# Autodesk Inventor assembly: Assembly1
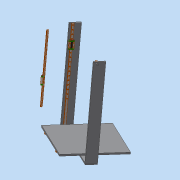
[picture p0: Inventor's stored thumbnail of the model, 180x180]
Saved by Autodesk Inventor 2016 (Build 200138000, 138)
## iProperties
Created: 2017-03-05
Part Number: Assembly1
Document SubType Name: Assembly
Designer: Errrm
Author: Errrm
## Documents named in this file (13)
- C:\Users\Lillahunden\Documents\Inventor\3dprinter\Assembly1.iam
- C:\Users\Lillahunden\Documents\Inventor\3dprinter\bed.ipt
- C:\Users\Lillahunden\Documents\Inventor\3dprinter\sideframe.ipt
- C:\Users\Lillahunden\Documents\Inventor\3dprinter\MGN7z.ipt
- C:\Users\Lillahunden\Documents\Inventor\3dprinter\MGN7x.ipt
- C:\Users\Lillahunden\Documents\Inventor\3dprinter\MGN7y.ipt
- C:\Users\Lillahunden\Documents\Inventor\3dprinter\MGN7-H.ipt
- C:\Users\Lillahunden\Documents\Inventor\3dprinter\bottomplate.ipt
- C:\Users\Lillahunden\Documents\Inventor\3dprinter\flat.ipt
- C:\Users\Lillahunden\Documents\Inventor\3dprinter\Angled foot.ipt
- C:\Users\Lillahunden\Documents\Inventor\3dprinter\Assembly1\Design Accelerator\Bolted Connection1.iam
- C:\Users\Lillahunden\Documents\Inventor\3dprinter\Assembly1\Design Accelerator\Bolted Connection2.iam
- C:\Users\Lillahunden\Documents\Inventor\Content Center Files\R2016\en-US\DIN 912\DIN 912 - M2 x 0,4 x 10 x 9.ipt
## Components (27 placed, 11 different names)
1. bed:1 — Mate:1, Mate:2, Mate:5, Mate:6, Flush:6, Angle:3, Mate:7, Flush:8, Flush:9
2. sideframe:1 — Flush:2, Flush:3, Mate:1, Mate:4, Flush:5, Mate:20
3. sideframe:2 — Flush:2, Flush:3, Mate:2, Mate:3, Angle:2, Flush:4, Angle:3, Flush:12, Flush:19, Flush:20
4. MGN7z:1 — Mate:4, Flush:5, Mate:12, Mate:13, Flush:16
5. MGN7z:2 — Mate:3, Angle:2, Flush:4, Mate:14, Mate:15, Flush:16
6. MGN7x:1 — Mate:16, Mate:17
7. MGN7y:1 — Mate:5, Mate:6, Flush:6, Flush:7, Flush:9, Angle:4, Mate:8, Mate:9
8. MGN7y:2 — Mate:7, Flush:7, Flush:8, Mate:10, Mate:11
9. MGN7-H:1 — Mate:12, Mate:13, Flush:11
10. MGN7-H:2 — Mate:14, Mate:15, Flush:11
11. MGN7-H:3 — Mate:16, Mate:17
12. MGN7-H:4 — Angle:4, Mate:8, Mate:9, Flush:10, Mate:19
13. MGN7-H:5 — Mate:10, Mate:11, Flush:10, Mate:18, Flush:21
14. bottomplate:1 — Flush:12, Mate:18, Mate:19, Angle:5, Mate:20, Flush:17, Mate:22, Flush:19, Flush:20, Flush:21, Mate:25, Mate:26, Mate:27, Mate:28, Insert:1, Insert:2, Insert:3, Insert:4, Insert:5, Insert:6, Insert:7, Insert:8
15. flat:1 — Flush:13, Angle:5
16. Angled foot:1 — Flush:17, Mate:21, Flush:18
17. Angled foot:2 — Mate:21, Mate:22, Flush:18
18. Bolted Connection:1 [sub-assembly] — Mate:27, Mate:28
19. Bolted Connection:2 [sub-assembly] — Mate:25, Mate:26
20. DIN 912 - replaced by DIN EN ISO 4762 M2 x 10:1 — Insert:1
21. DIN 912 - replaced by DIN EN ISO 4762 M2 x 10:2 — Insert:2
22. DIN 912 - replaced by DIN EN ISO 4762 M2 x 10:3 — Insert:3
23. DIN 912 - replaced by DIN EN ISO 4762 M2 x 10:4 — Insert:4
24. DIN 912 - replaced by DIN EN ISO 4762 M2 x 10:5 — Insert:5
25. DIN 912 - replaced by DIN EN ISO 4762 M2 x 10:6 — Insert:6
26. DIN 912 - replaced by DIN EN ISO 4762 M2 x 10:7 — Insert:7
27. DIN 912 - replaced by DIN EN ISO 4762 M2 x 10:8 — Insert:8
## Relationships (56: Mate 26, Flush 18, Insert 8, Angle 4)
- Flush:2: sideframe:1 ↔ sideframe:2
- Flush:3: sideframe:1 ↔ sideframe:2
- Mate:1 (35 mm): bed:1 ↔ sideframe:1
- Mate:2 (35 mm): bed:1 ↔ sideframe:2
- Mate:3: sideframe:2 ↔ MGN7z:2
- Mate:4: sideframe:1 ↔ MGN7z:1
- Angle:2 (0 deg): sideframe:2 ↔ MGN7z:2
- Flush:4: sideframe:2 ↔ MGN7z:2
- Flush:5: sideframe:1 ↔ MGN7z:1
- Mate:5: bed:1 ↔ MGN7y:1
- Mate:6: bed:1 ↔ MGN7y:1
- Flush:6: bed:1 ↔ MGN7y:1
- Angle:3 (0 deg): bed:1 ↔ sideframe:2
- Mate:7: bed:1 ↔ MGN7y:2
- Flush:7: MGN7y:1 ↔ MGN7y:2
- Flush:8 (38 mm): bed:1 ↔ MGN7y:2
- Flush:9 (38 mm): bed:1 ↔ MGN7y:1
- Angle:4 (0 deg): MGN7y:1 ↔ MGN7-H:4
- Mate:8: MGN7y:1 ↔ MGN7-H:4
- Mate:9: MGN7y:1 ↔ MGN7-H:4
- Mate:10: MGN7y:2 ↔ MGN7-H:5
- Mate:11: MGN7y:2 ↔ MGN7-H:5
- Flush:10: MGN7-H:4 ↔ MGN7-H:5
- Mate:12: MGN7z:1 ↔ MGN7-H:1
- Mate:13: MGN7z:1 ↔ MGN7-H:1
- Mate:14: MGN7z:2 ↔ MGN7-H:2
- Mate:15: MGN7z:2 ↔ MGN7-H:2
- Flush:11: MGN7-H:1 ↔ MGN7-H:2
- Mate:16: MGN7x:1 ↔ MGN7-H:3
- Mate:17: MGN7x:1 ↔ MGN7-H:3
- Flush:12: sideframe:2 ↔ bottomplate:1
- Mate:18: MGN7-H:5 ↔ bottomplate:1
- Mate:19: MGN7-H:4 ↔ bottomplate:1
- Flush:13: flat:1
- Angle:5 (0 deg): bottomplate:1 ↔ flat:1
- Mate:20: sideframe:1 ↔ bottomplate:1
- Flush:16: MGN7z:1 ↔ MGN7z:2
- Flush:17: bottomplate:1 ↔ Angled foot:1
- Mate:21: Angled foot:1 ↔ Angled foot:2
- Mate:22: bottomplate:1 ↔ Angled foot:2
- Flush:18: Angled foot:1 ↔ Angled foot:2
- Flush:19: sideframe:2 ↔ bottomplate:1
- Flush:20: sideframe:2 ↔ bottomplate:1
- Flush:21 (3.6 mm): MGN7-H:5 ↔ bottomplate:1
- Mate:25: bottomplate:1 ↔ Bolted Connection:2
- Mate:26: bottomplate:1 ↔ Bolted Connection:2
- Mate:27: bottomplate:1 ↔ Bolted Connection:1
- Mate:28: bottomplate:1 ↔ Bolted Connection:1
- Insert:1: bottomplate:1 ↔ DIN 912 - replaced by DIN EN ISO 4762 M2 x 10:1
- Insert:2: bottomplate:1 ↔ DIN 912 - replaced by DIN EN ISO 4762 M2 x 10:2
- Insert:3: bottomplate:1 ↔ DIN 912 - replaced by DIN EN ISO 4762 M2 x 10:3
- Insert:4: bottomplate:1 ↔ DIN 912 - replaced by DIN EN ISO 4762 M2 x 10:4
- Insert:5: bottomplate:1 ↔ DIN 912 - replaced by DIN EN ISO 4762 M2 x 10:5
- Insert:6: bottomplate:1 ↔ DIN 912 - replaced by DIN EN ISO 4762 M2 x 10:6
- Insert:7: bottomplate:1 ↔ DIN 912 - replaced by DIN EN ISO 4762 M2 x 10:7
- Insert:8: bottomplate:1 ↔ DIN 912 - replaced by DIN EN ISO 4762 M2 x 10:8
